# Autodesk Inventor assembly: Assemble
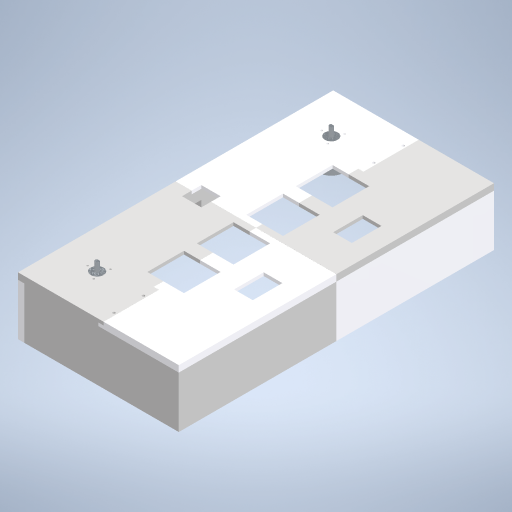
[picture p0: Inventor's stored thumbnail of the model, 512x512]
Saved by Autodesk Inventor 2023 (Build 270158000, 158)
## iProperties
Created: 2024-04-26
Part Number: Assemble
Document SubType Name: Assembly
Designer: Nitrene.P.L
Author: Nitrene.P.L
## Documents named in this file (12)
- E:\Github\AgSDVX\Case\Assemble.iam
- E:\Github\AgSDVX\Case\top_1.ipt
- E:\Github\AgSDVX\Case\top_2.ipt
- E:\Github\AgSDVX\Case\top_3.ipt
- E:\Github\AgSDVX\Case\top_4.ipt
- E:\Github\AgSDVX\Case\front_1.ipt
- E:\Github\AgSDVX\Case\front_2.ipt
- E:\Github\AgSDVX\Case\left.ipt
- E:\Github\AgSDVX\Case\right.ipt
- E:\Github\AgSDVX\Case\back_1.ipt
- E:\Github\AgSDVX\Case\back_2.ipt
- E:\Github\AgSDVX\Case\rotary_encoder.ipt
## Components (12 placed, 11 different names)
1. top_1:1 — 配合:1, 表面齐平:1, 表面齐平:2, 配合:3, 表面齐平:5, 表面齐平:6, 配合:11, 插入:1
2. top_2:1 — 配合:1, 表面齐平:1, 表面齐平:2, 配合:2, 表面齐平:3, 表面齐平:4, 配合:8, 配合:14, 插入:2
3. top_3:1 — 配合:3, 表面齐平:5, 表面齐平:6, 配合:4, 表面齐平:7, 表面齐平:8, 配合:6
4. top_4:1 — 配合:2, 表面齐平:3, 表面齐平:4, 配合:5, 表面齐平:9, 表面齐平:10, 表面齐平:12
5. front_1:1 — 配合:5, 表面齐平:9, 表面齐平:10, 配合:9, 配合:10
6. front_2:1 — 配合:4, 表面齐平:7, 表面齐平:8, 表面齐平:11, 配合:7
7. left:1 — 配合:6, 表面齐平:11, 配合:7, 配合:12, 表面齐平:13
8. right:1 — 表面齐平:12, 配合:8, 配合:9, 配合:10, 配合:15
9. back_1:1 — 配合:11, 配合:12, 表面齐平:13, 配合:13
10. back_2:1 — 配合:13, 配合:14, 配合:15
11. rotary_encoder:1 — 插入:1
12. rotary_encoder:2 — 插入:2
## Relationships (30: Mate 15, Flush 13, Insert 2)
- 配合:1 [Mate]: top_1:1 ↔ top_2:1
- 表面齐平:1 [Flush]: top_1:1 ↔ top_2:1
- 表面齐平:2 [Flush]: top_1:1 ↔ top_2:1
- 配合:2 [Mate]: top_2:1 ↔ top_4:1
- 表面齐平:3 [Flush]: top_2:1 ↔ top_4:1
- 表面齐平:4 [Flush]: top_2:1 ↔ top_4:1
- 配合:3 [Mate]: top_1:1 ↔ top_3:1
- 表面齐平:5 [Flush]: top_1:1 ↔ top_3:1
- 表面齐平:6 [Flush]: top_1:1 ↔ top_3:1
- 配合:4 [Mate]: top_3:1 ↔ front_2:1
- 表面齐平:7 [Flush]: top_3:1 ↔ front_2:1
- 表面齐平:8 [Flush]: top_3:1 ↔ front_2:1
- 配合:5 [Mate]: top_4:1 ↔ front_1:1
- 表面齐平:9 [Flush]: top_4:1 ↔ front_1:1
- 表面齐平:10 [Flush]: top_4:1 ↔ front_1:1
- 配合:6 [Mate]: top_3:1 ↔ left:1
- 表面齐平:11 [Flush]: front_2:1 ↔ left:1
- 配合:7 [Mate]: front_2:1 ↔ left:1
- 表面齐平:12 [Flush]: top_4:1 ↔ right:1
- 配合:8 [Mate]: top_2:1 ↔ right:1
- 配合:9 [Mate]: front_1:1 ↔ right:1
- 配合:10 [Mate]: front_1:1 ↔ right:1
- 配合:11 [Mate]: top_1:1 ↔ back_1:1
- 配合:12 [Mate]: left:1 ↔ back_1:1
- 表面齐平:13 [Flush]: left:1 ↔ back_1:1
- 配合:13 [Mate]: back_1:1 ↔ back_2:1
- 配合:14 [Mate]: top_2:1 ↔ back_2:1
- 配合:15 [Mate]: right:1 ↔ back_2:1
- 插入:1 [Insert]: top_1:1 ↔ rotary_encoder:1
- 插入:2 [Insert]: top_2:1 ↔ rotary_encoder:2
